# Autodesk Inventor assembly: gear_box_base
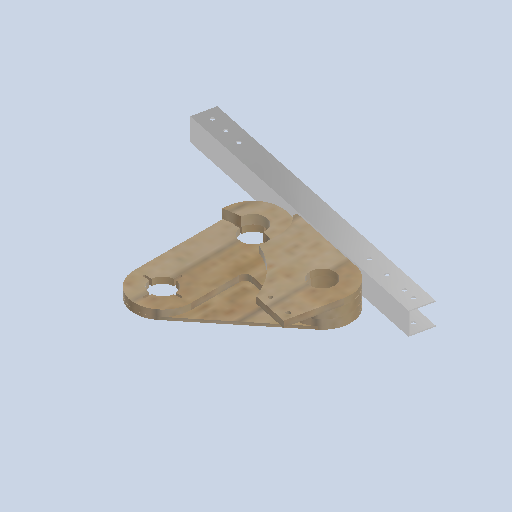
[picture p0: Inventor's stored thumbnail of the model, 512x512]
Saved by Autodesk Inventor 2024.1 (Build 281209000, 209)
## iProperties
Created: 2025-09-25
Part Number: gear_box_base
Document SubType Name: Assembly
Designer: hibik
Author: hibik
## Documents named in this file (6)
- C:\Users\hibik\Documents\Robomech\conveyer\power_module\gear_box_base.iam
- C:\Users\hibik\Documents\Robomech\conveyer\power_module\gear_plate_1.ipt
- C:\Users\hibik\Documents\Robomech\conveyer\power_module\gear_plate_2.ipt
- C:\Users\hibik\Documents\Robomech\conveyer\power_module\gear_plate_3.ipt
- C:\Users\hibik\Documents\Robomech\conveyer\power_module\gear_plate_base.ipt
- C:\Users\hibik\Documents\Robomech\conveyer\power_module\gear_plate_pole.ipt
## Components (5 placed, 5 different names)
1. gear_plate_1:1 — 挿入:1, 挿入:2, 挿入:5, 挿入:6
2. gear_plate_2:1 — 挿入:1, 挿入:2, 挿入:3, 挿入:4
3. gear_plate_3:1 — 挿入:3, 挿入:4, 角度:1
4. gear_plate_base:1 — 挿入:5, 挿入:6, 挿入:7
5. gear_plate_pole:1 — 挿入:7, 角度:1
## Relationships (8: Insert 7, Angle 1)
- 挿入:1 [Insert]: gear_plate_1:1 ↔ gear_plate_2:1
- 挿入:2 [Insert]: gear_plate_1:1 ↔ gear_plate_2:1
- 挿入:3 [Insert]: gear_plate_2:1 ↔ gear_plate_3:1
- 挿入:4 [Insert]: gear_plate_2:1 ↔ gear_plate_3:1
- 挿入:5 [Insert]: gear_plate_1:1 ↔ gear_plate_base:1
- 挿入:6 [Insert]: gear_plate_1:1 ↔ gear_plate_base:1
- 挿入:7 [Insert]: gear_plate_base:1 ↔ gear_plate_pole:1
- 角度:1 [Angle] (180 deg): gear_plate_3:1 ↔ gear_plate_pole:1
